# Autodesk Inventor assembly: Assembly6
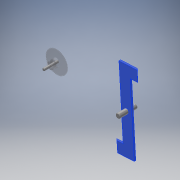
[picture p0: Inventor's stored thumbnail of the model, 180x180]
Saved by Autodesk Inventor 2017 (Build 210142000, 142)
## iProperties
Created: 2016-12-06
Part Number: Assembly6
Document SubType Name: Assembly
Designer: aesen
Author: aesen
## Documents named in this file (7)
- C:\Users\aesen\Design\newassembly\W1chain\Assembly6.iam
- C:\Users\aesen\Design\newassembly\W1chain\2737T522_FINISHED-BORE SPROCKET FOR ANSI ROLLER CHAIN.ipt
- C:\Users\aesen\Design\newassembly\W1chain\62375K110_QUICK-DISCONNECT BUSHING-BORE SPROCKET.ipt
- C:\Users\aesen\Design\newassembly\W1chain\6529K250_MTL MITER GEAR--20 DEG PRESSURE ANGLE.ipt
- C:\Users\aesen\Design\newassembly\W1chain\Assembly6\Design Accelerator\Shaft1.iam
- C:\Users\aesen\Design\newassembly\W1chain\Blunt_Blade.0003.ipt
- C:\Users\aesen\Design\newassembly\W1chain\Assembly6\Design Accelerator\Shaft4.iam
## Components (6 placed, 5 different names)
1. 62375K110_QUICK-DISCONNECT BUSHING-BORE SPROCKET:1 — Insert:1
2. 6529K250_MTL MITER GEAR--20 DEG PRESSURE ANGLE:1 — Insert:4
3. Shaft:1 [sub-assembly] — Insert:1, Insert:2
4. Blunt_Blade.0003:1 — Insert:2
5. Shaft:2 [sub-assembly] — Insert:4, Insert:5
6. 2737T522_FINISHED-BORE SPROCKET FOR ANSI ROLLER CHAIN:1 — Insert:5
## Relationships (4: Insert 4)
- Insert:1 (-50.8 mm): 62375K110_QUICK-DISCONNECT BUSHING-BORE SPROCKET:1 ↔ Shaft:1
- Insert:2 (-66.04 mm): Shaft:1 ↔ Blunt_Blade.0003:1
- Insert:4 (-76.2 mm): 6529K250_MTL MITER GEAR--20 DEG PRESSURE ANGLE:1 ↔ Shaft:2
- Insert:5 (-31.75 mm): Shaft:2 ↔ 2737T522_FINISHED-BORE SPROCKET FOR ANSI ROLLER CHAIN:1
